# Autodesk Inventor assembly: post
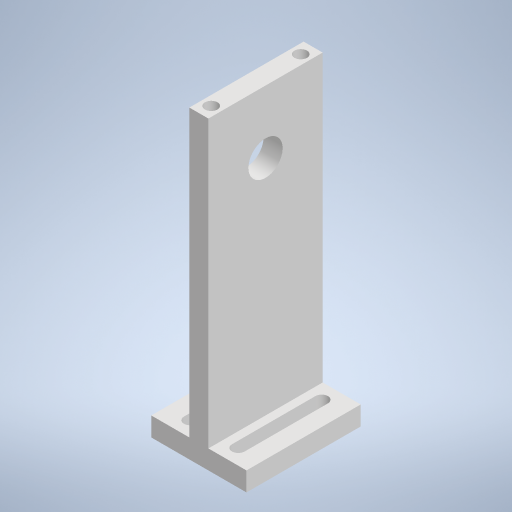
[picture p0: Inventor's stored thumbnail of the model, 512x512]
Saved by Autodesk Inventor 2024 (Build 280153000, 153)
## iProperties
Created: 2024-11-05
Part Number: post
Document SubType Name: Assembly
Designer: Andreas Weber
Author: Andreas Weber
## Documents named in this file (4)
- C:\Users\Andreas Weber\Desktop\Upload for Github\post.iam
- C:\Users\Andreas Weber\Desktop\Upload for Github\post_base.ipt
- C:\Users\Andreas Weber\Desktop\Upload for Github\post_bottom.ipt
- C:\Users\Andreas Weber\Desktop\Upload for Github\post_top.ipt
## Components (3 placed, 3 different names)
1. post_base:1 — Starr:1
2. post_bottom:1 — Starr:1, Drehbar:1
3. post_top:1 — Drehbar:1
## Relationships (2: WeldJoint 1, RevoluteJoint 1)
- Starr:1 [WeldJoint]: post_base:1 ↔ post_bottom:1
- Drehbar:1 [RevoluteJoint]: post_bottom:1 ↔ post_top:1
